# Autodesk Inventor assembly: FInny's assembly
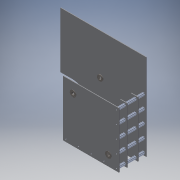
[picture p0: Inventor's stored thumbnail of the model, 180x180]
Saved by Autodesk Inventor 2016 (Build 200138000, 138)
## iProperties
Created: 2017-01-29
Part Number: FInny's assembly
Document SubType Name: Assembly
Designer: rasmussenf
Author: rasmussenf
## Documents named in this file (7)
- E:\1073CAD\Robot2017\Parts\FInny's assembly.iam
- Z:\IED\CAD\Shooter 2017\1073-2017 Shooter Outside Plate Right.ipt
- Z:\IED\CAD\Shooter 2017\1073-2017 Shooter Inside Plate.ipt
- E:\1073CAD\Robot2017\Parts\1,5InchChurro.ipt
- E:\1073CAD\Robot2017\Parts\2InchChurro.ipt
- Z:\IED\CAD\Shooter 2017\1073-2017 Shooter Outside Plate Left.ipt
- E:\1073CAD\Robot2017\VEXpro-CAD-Files-20170103\Motion\Bearings\217-3875-STEP-20140818.ipt
## Components (35 placed, 6 different names)
1. 1073-2017 Shooter Outside Plate Right:1 — Flush:1, Flush:2, Mate:1, Mate:2, Mate:4, Mate:6, Mate:8, Mate:11, Mate:12, Mate:14, Mate:16, Mate:18, Mate:58, Mate:59, Mate:62, Mate:63
2. 1073-2017 Shooter Inside Plate:1 — Flush:1, Flush:2, Mate:1, Mate:3, Mate:5, Mate:7, Mate:9, Mate:10, Mate:13, Mate:15, Mate:17, Mate:19, Flush:3, Flush:4, Mate:20, Mate:21, Mate:23, Mate:25, Mate:27, Mate:29, Mate:31, Mate:33, Mate:35, Mate:37
3. 1,5InchChurro:1 — Mate:2, Mate:3
4. 1,5InchChurro:2 — Mate:4, Mate:5
5. 1,5InchChurro:3 — Mate:6, Mate:7
6. 1,5InchChurro:4 — Mate:8, Mate:9
7. 1,5InchChurro:5 — Mate:10, Mate:11
8. 1,5InchChurro:6 — Mate:12, Mate:13
9. 1,5InchChurro:7 — Mate:14, Mate:15
10. 1,5InchChurro:8 — Mate:16, Mate:17
11. 1,5InchChurro:9 — Mate:18, Mate:19
12. 1073-2017 Shooter Inside Plate:2 — Flush:3, Flush:4, Mate:20, Mate:22, Mate:24, Mate:26, Mate:28, Mate:30, Mate:32, Mate:34, Mate:36, Mate:38, Flush:5, Flush:6, Mate:39, Mate:40, Mate:42, Mate:44, Mate:46, Mate:48, Mate:50, Mate:52, Mate:54, Mate:56
13. 2InchChurro:1 — Mate:21, Mate:22
14. 2InchChurro:2 — Mate:23, Mate:24
15. 2InchChurro:3 — Mate:25, Mate:26
16. 2InchChurro:4 — Mate:27, Mate:28
17. 2InchChurro:5 — Mate:29, Mate:30
18. 2InchChurro:6 — Mate:31, Mate:32
19. 2InchChurro:7 — Mate:33, Mate:34
20. 2InchChurro:8 — Mate:35, Mate:36
21. 2InchChurro:9 — Mate:37, Mate:38
22. 1073-2017 Shooter Outside Plate Left:1 — Flush:5, Flush:6, Mate:39, Mate:41, Mate:43, Mate:45, Mate:47, Mate:49, Mate:51, Mate:53, Mate:55, Mate:57, Mate:60, Mate:61, Mate:64, Mate:65
23. 1,5InchChurro:10 — Mate:40, Mate:41
24. 1,5InchChurro:11 — Mate:42, Mate:43
25. 1,5InchChurro:12 — Mate:44, Mate:45
26. 1,5InchChurro:13 — Mate:46, Mate:47
27. 1,5InchChurro:14 — Mate:48, Mate:49
28. 1,5InchChurro:15 — Mate:50, Mate:51
29. 1,5InchChurro:16 — Mate:52, Mate:53
30. 1,5InchChurro:17 — Mate:54, Mate:55
31. 1,5InchChurro:18 — Mate:56, Mate:57
32. 217-3875-STEP-20140818:1 — Mate:58, Mate:59
33. 217-3875-STEP-20140818:2 — Mate:60, Mate:61
34. 217-3875-STEP-20140818:3 — Mate:62, Mate:63
35. 217-3875-STEP-20140818:4 — Mate:64, Mate:65
## Relationships (71: Mate 65, Flush 6)
- Flush:1: 1073-2017 Shooter Outside Plate Right:1 ↔ 1073-2017 Shooter Inside Plate:1
- Flush:2: 1073-2017 Shooter Outside Plate Right:1 ↔ 1073-2017 Shooter Inside Plate:1
- Mate:1 (38.1 mm): 1073-2017 Shooter Outside Plate Right:1 ↔ 1073-2017 Shooter Inside Plate:1
- Mate:2: 1073-2017 Shooter Outside Plate Right:1 ↔ 1,5InchChurro:1
- Mate:3: 1073-2017 Shooter Inside Plate:1 ↔ 1,5InchChurro:1
- Mate:4: 1073-2017 Shooter Outside Plate Right:1 ↔ 1,5InchChurro:2
- Mate:5: 1073-2017 Shooter Inside Plate:1 ↔ 1,5InchChurro:2
- Mate:6: 1073-2017 Shooter Outside Plate Right:1 ↔ 1,5InchChurro:3
- Mate:7: 1073-2017 Shooter Inside Plate:1 ↔ 1,5InchChurro:3
- Mate:8: 1073-2017 Shooter Outside Plate Right:1 ↔ 1,5InchChurro:4
- Mate:9: 1073-2017 Shooter Inside Plate:1 ↔ 1,5InchChurro:4
- Mate:10: 1073-2017 Shooter Inside Plate:1 ↔ 1,5InchChurro:5
- Mate:11: 1073-2017 Shooter Outside Plate Right:1 ↔ 1,5InchChurro:5
- Mate:12: 1073-2017 Shooter Outside Plate Right:1 ↔ 1,5InchChurro:6
- Mate:13: 1073-2017 Shooter Inside Plate:1 ↔ 1,5InchChurro:6
- Mate:14: 1073-2017 Shooter Outside Plate Right:1 ↔ 1,5InchChurro:7
- Mate:15: 1073-2017 Shooter Inside Plate:1 ↔ 1,5InchChurro:7
- Mate:16: 1073-2017 Shooter Outside Plate Right:1 ↔ 1,5InchChurro:8
- Mate:17: 1073-2017 Shooter Inside Plate:1 ↔ 1,5InchChurro:8
- Mate:18: 1073-2017 Shooter Outside Plate Right:1 ↔ 1,5InchChurro:9
- Mate:19: 1073-2017 Shooter Inside Plate:1 ↔ 1,5InchChurro:9
- Flush:3: 1073-2017 Shooter Inside Plate:1 ↔ 1073-2017 Shooter Inside Plate:2
- Flush:4: 1073-2017 Shooter Inside Plate:1 ↔ 1073-2017 Shooter Inside Plate:2
- Mate:20 (50.8 mm): 1073-2017 Shooter Inside Plate:1 ↔ 1073-2017 Shooter Inside Plate:2
- Mate:21: 1073-2017 Shooter Inside Plate:1 ↔ 2InchChurro:1
- Mate:22: 1073-2017 Shooter Inside Plate:2 ↔ 2InchChurro:1
- Mate:23: 1073-2017 Shooter Inside Plate:1 ↔ 2InchChurro:2
- Mate:24: 1073-2017 Shooter Inside Plate:2 ↔ 2InchChurro:2
- Mate:25: 1073-2017 Shooter Inside Plate:1 ↔ 2InchChurro:3
- Mate:26: 1073-2017 Shooter Inside Plate:2 ↔ 2InchChurro:3
- Mate:27: 1073-2017 Shooter Inside Plate:1 ↔ 2InchChurro:4
- Mate:28: 1073-2017 Shooter Inside Plate:2 ↔ 2InchChurro:4
- Mate:29: 1073-2017 Shooter Inside Plate:1 ↔ 2InchChurro:5
- Mate:30: 1073-2017 Shooter Inside Plate:2 ↔ 2InchChurro:5
- Mate:31: 1073-2017 Shooter Inside Plate:1 ↔ 2InchChurro:6
- Mate:32: 1073-2017 Shooter Inside Plate:2 ↔ 2InchChurro:6
- Mate:33: 1073-2017 Shooter Inside Plate:1 ↔ 2InchChurro:7
- Mate:34: 1073-2017 Shooter Inside Plate:2 ↔ 2InchChurro:7
- Mate:35: 1073-2017 Shooter Inside Plate:1 ↔ 2InchChurro:8
- Mate:36: 1073-2017 Shooter Inside Plate:2 ↔ 2InchChurro:8
- Mate:37: 1073-2017 Shooter Inside Plate:1 ↔ 2InchChurro:9
- Mate:38: 1073-2017 Shooter Inside Plate:2 ↔ 2InchChurro:9
- Flush:5: 1073-2017 Shooter Inside Plate:2 ↔ 1073-2017 Shooter Outside Plate Left:1
- Flush:6: 1073-2017 Shooter Inside Plate:2 ↔ 1073-2017 Shooter Outside Plate Left:1
- Mate:39 (38.1 mm): 1073-2017 Shooter Inside Plate:2 ↔ 1073-2017 Shooter Outside Plate Left:1
- Mate:40: 1073-2017 Shooter Inside Plate:2 ↔ 1,5InchChurro:10
- Mate:41: 1073-2017 Shooter Outside Plate Left:1 ↔ 1,5InchChurro:10
- Mate:42: 1073-2017 Shooter Inside Plate:2 ↔ 1,5InchChurro:11
- Mate:43: 1073-2017 Shooter Outside Plate Left:1 ↔ 1,5InchChurro:11
- Mate:44: 1073-2017 Shooter Inside Plate:2 ↔ 1,5InchChurro:12
- Mate:45: 1073-2017 Shooter Outside Plate Left:1 ↔ 1,5InchChurro:12
- Mate:46: 1073-2017 Shooter Inside Plate:2 ↔ 1,5InchChurro:13
- Mate:47: 1073-2017 Shooter Outside Plate Left:1 ↔ 1,5InchChurro:13
- Mate:48: 1073-2017 Shooter Inside Plate:2 ↔ 1,5InchChurro:14
- Mate:49: 1073-2017 Shooter Outside Plate Left:1 ↔ 1,5InchChurro:14
- Mate:50: 1073-2017 Shooter Inside Plate:2 ↔ 1,5InchChurro:15
- Mate:51: 1073-2017 Shooter Outside Plate Left:1 ↔ 1,5InchChurro:15
- Mate:52: 1073-2017 Shooter Inside Plate:2 ↔ 1,5InchChurro:16
- Mate:53: 1073-2017 Shooter Outside Plate Left:1 ↔ 1,5InchChurro:16
- Mate:54: 1073-2017 Shooter Inside Plate:2 ↔ 1,5InchChurro:17
- Mate:55: 1073-2017 Shooter Outside Plate Left:1 ↔ 1,5InchChurro:17
- Mate:56: 1073-2017 Shooter Inside Plate:2 ↔ 1,5InchChurro:18
- Mate:57: 1073-2017 Shooter Outside Plate Left:1 ↔ 1,5InchChurro:18
- Mate:58: 1073-2017 Shooter Outside Plate Right:1 ↔ 217-3875-STEP-20140818:1
- Mate:59: 1073-2017 Shooter Outside Plate Right:1 ↔ 217-3875-STEP-20140818:1
- Mate:60: 1073-2017 Shooter Outside Plate Left:1 ↔ 217-3875-STEP-20140818:2
- Mate:61: 1073-2017 Shooter Outside Plate Left:1 ↔ 217-3875-STEP-20140818:2
- Mate:62: 1073-2017 Shooter Outside Plate Right:1 ↔ 217-3875-STEP-20140818:3
- Mate:63: 1073-2017 Shooter Outside Plate Right:1 ↔ 217-3875-STEP-20140818:3
- Mate:64: 1073-2017 Shooter Outside Plate Left:1 ↔ 217-3875-STEP-20140818:4
- Mate:65: 1073-2017 Shooter Outside Plate Left:1 ↔ 217-3875-STEP-20140818:4
